# Autodesk Inventor assembly: Pi Cam and Cable assembly
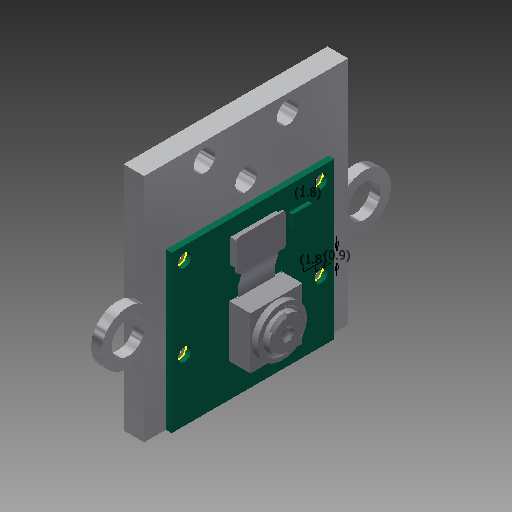
[picture p0: Inventor's stored thumbnail of the model, 512x512]
Saved by Autodesk Inventor 2017 (Build 210142000, 142)
## iProperties
Created: 2017-01-19
Part Number: Pi Cam and Cable assembly
Document SubType Name: Assembly
Designer: qupec
Author: qupec
## Documents named in this file (4)
- C:\Users\qupec\Desktop\UMD Near Space\RockSat\Pi Cam and Cable assembly.iam
- C:\Users\qupec\Desktop\UMD Near Space\RockSat\Pi Cam\RasPi_Camera.iam
- C:\Users\qupec\Desktop\UMD Near Space\RockSat\Ribbon Cable Connector-01.ipt
- C:\Users\qupec\Desktop\UMD Near Space\RockSat\Pi cCam Mount.ipt
## Components (3 placed, 3 different names)
1. RasPi_Camera:1 [sub-assembly] — Mate:1, Flush:1, Flush:2, Mate:2, Mate:3, Mate:4
2. Ribbon Cable Connector-01:2 — Mate:1, Flush:1, Flush:2
3. Pi cCam Mount:1 — Mate:2, Mate:3, Mate:4
## Relationships (6: Mate 4, Flush 2)
- Mate:1: RasPi_Camera:1 ↔ Ribbon Cable Connector-01:2
- Flush:1 (2.1 mm): RasPi_Camera:1 ↔ Ribbon Cable Connector-01:2
- Flush:2: RasPi_Camera:1 ↔ Ribbon Cable Connector-01:2
- Mate:2: RasPi_Camera:1 ↔ Pi cCam Mount:1
- Mate:3: RasPi_Camera:1 ↔ Pi cCam Mount:1
- Mate:4: RasPi_Camera:1 ↔ Pi cCam Mount:1
